# Autodesk Inventor assembly: Durometer_Slide_Fixture
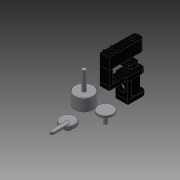
[picture p0: Inventor's stored thumbnail of the model, 180x180]
Saved by Autodesk Inventor 2015 (Build 190159000, 159)
## iProperties
Created: 2014-12-16
Part Number: Durometer_Slide_Fixture
Document SubType Name: Assembly
Designer: amarschn
Author: amarschn
## Documents named in this file (12)
- \\andrew.ad.cmu.edu\users\users7\amarschn\Documents\Durometer_Assembly\Durometer_Slide_Fixture.iam
- \\andrew.ad.cmu.edu\users\users7\amarschn\Documents\Durometer_Assembly\Fixture_Base.ipt
- \\andrew.ad.cmu.edu\users\users7\amarschn\Documents\Durometer_Assembly\Fixture_Base_Support.ipt
- \\andrew.ad.cmu.edu\users\users7\amarschn\Documents\Durometer_Assembly\Fixture_Airpot_Support.ipt
- \\andrew.ad.cmu.edu\users\users7\amarschn\Documents\Durometer_Assembly\Fixture_Airpot_Support_2.ipt
- \\andrew.ad.cmu.edu\users\users7\amarschn\Documents\Durometer_Assembly\Fixture_Airpot_Support_3.ipt
- \\andrew.ad.cmu.edu\users\users7\amarschn\Documents\Durometer_Assembly\Fixture_Airpot.ipt
- \\andrew.ad.cmu.edu\users\users7\amarschn\Documents\Durometer_Assembly\Fixture_Slide_Lock_Plate.ipt
- \\andrew.ad.cmu.edu\users\users7\amarschn\Documents\Durometer_Assembly\Fixture_Weight.ipt
- \\andrew.ad.cmu.edu\users\users7\amarschn\Documents\Durometer_Assembly\Fixture_Knob_1.ipt
- \\andrew.ad.cmu.edu\users\users7\amarschn\Documents\Durometer_Assembly\Fixture_Knob_2.ipt
- \\andrew.ad.cmu.edu\users\users7\amarschn\Documents\Durometer_Assembly\Fixture_Lever.ipt
## Components (11 placed, 11 different names)
1. Fixture_Base:1 — Mate:1, Flush:1, Flush:2, Mate:2
2. Fixture_Base_Support:1 — Mate:1, Flush:1, Flush:2, Mate:3, Flush:7
3. Fixture_Airpot_Support:1 — Mate:2, Mate:3, Mate:4, Flush:3, Flush:4, Mate:6, Flush:7
4. Fixture_Airpot_Support_2:1 — Mate:5, Flush:5, Flush:6, Mate:7
5. Fixture_Airpot_Support_3:1 — Mate:4, Flush:3, Flush:4, Mate:5, Flush:5, Flush:6
6. Fixture_Airpot:1 — Mate:6, Mate:7
7. Fixture_Slide_Lock_Plate:1
8. Fixture_Weight:1
9. Fixture_Knob_1:1
10. Fixture_Knob_2:1
11. Fixture_Lever:1
## Relationships (14: Mate 7, Flush 7)
- Mate:1: Fixture_Base:1 ↔ Fixture_Base_Support:1
- Flush:1: Fixture_Base:1 ↔ Fixture_Base_Support:1
- Flush:2: Fixture_Base:1 ↔ Fixture_Base_Support:1
- Mate:2: Fixture_Base:1 ↔ Fixture_Airpot_Support:1
- Mate:3: Fixture_Base_Support:1 ↔ Fixture_Airpot_Support:1
- Mate:4: Fixture_Airpot_Support:1 ↔ Fixture_Airpot_Support_3:1
- Flush:3: Fixture_Airpot_Support:1 ↔ Fixture_Airpot_Support_3:1
- Flush:4: Fixture_Airpot_Support:1 ↔ Fixture_Airpot_Support_3:1
- Mate:5: Fixture_Airpot_Support_2:1 ↔ Fixture_Airpot_Support_3:1
- Flush:5: Fixture_Airpot_Support_2:1 ↔ Fixture_Airpot_Support_3:1
- Flush:6: Fixture_Airpot_Support_2:1 ↔ Fixture_Airpot_Support_3:1
- Mate:6: Fixture_Airpot_Support:1 ↔ Fixture_Airpot:1
- Mate:7: Fixture_Airpot_Support_2:1 ↔ Fixture_Airpot:1
- Flush:7: Fixture_Base_Support:1 ↔ Fixture_Airpot_Support:1
